# Autodesk Inventor assembly: RobotMK1
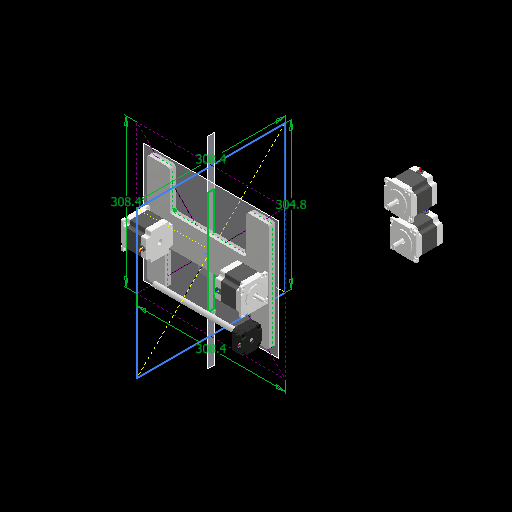
[picture p0: Inventor's stored thumbnail of the model, 512x512]
Saved by Autodesk Inventor 2025 (Build 290162000, 162)
## iProperties
Created: 2024-11-11
Part Number: RobotMK1
Document SubType Name: Assembly
Designer: Trevor
Author: Trevor
## Documents named in this file (6)
- C:\Users\Trevor\Documents\GitHub\USA-Robotic-Club-2024\assests\RobotMK1.iam
- C:\Users\Trevor\Documents\GitHub\USA-Robotic-Club-2024\assests\Newest base v1.ipt
- C:\Users\Trevor\Documents\GitHub\USA-Robotic-Club-2024\assests\stepper-motor-nema-23-57bygh201-1.snapshot.3\nema23_57byg201\nema23_57byg201.ipt
- C:\Users\Trevor\Documents\GitHub\USA-Robotic-Club-2024\assests\17hm08-1204s-nema17-pancake-21mm-1.snapshot.2\17HM08-1204S Nema17 Pancake 21mm\17HM08-1204S Nema17 Pancake 21mm.ipt
- C:\Users\Trevor\Documents\GitHub\USA-Robotic-Club-2024\assests\Part147.ipt
- C:\Users\Trevor\Documents\GitHub\USA-Robotic-Club-2024\assests\Part148.ipt
## Components (9 placed, 5 different names)
1. Newest base v1:1 — Mate:1, Flush:1, Mate:2, Flush:2, Mate:3, Flush:3, Flush:4
2. nema23_57byg201:1 — Mate:1, Flush:1, Flush:6
3. nema23_57byg201:2
4. nema23_57byg201:3
5. nema23_57byg201:4 — Mate:2, Flush:2
6. 17HM08-1204S Nema17 Pancake 21mm:1 — Mate:3, Flush:3, Flush:4, Flush:5
7. 17HM08-1204S Nema17 Pancake 21mm:2
8. Part147:1 — Flush:5
9. Part148:1 — Flush:6
## Relationships (9: Flush 6, Mate 3)
- Mate:1: Newest base v1:1 ↔ nema23_57byg201:1
- Flush:1: Newest base v1:1 ↔ nema23_57byg201:1
- Mate:2: Newest base v1:1 ↔ nema23_57byg201:4
- Flush:2: Newest base v1:1 ↔ nema23_57byg201:4
- Mate:3: Newest base v1:1 ↔ 17HM08-1204S Nema17 Pancake 21mm:1
- Flush:3: Newest base v1:1 ↔ 17HM08-1204S Nema17 Pancake 21mm:1
- Flush:4: Newest base v1:1 ↔ 17HM08-1204S Nema17 Pancake 21mm:1
- Flush:5: 17HM08-1204S Nema17 Pancake 21mm:1 ↔ Part147:1
- Flush:6: nema23_57byg201:1 ↔ Part148:1
